# Autodesk Inventor assembly: Piston
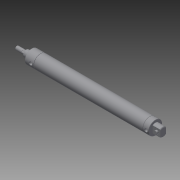
[picture p0: Inventor's stored thumbnail of the model, 180x180]
Saved by Autodesk Inventor 2014 (Build 180170000, 170)
## iProperties
Created: 2014-01-08
Part Number: Piston
Document SubType Name: Assembly
Designer: Tristan Debrunner
Author: Tristan Debrunner
## Documents named in this file (6)
- C:\Users\Tristan Debrunner\Documents\FRC 2014\Chassis\Piston.iam
- C:\Users\Tristan Debrunner\Documents\Inventor\Part2.ipt
- C:\Users\Tristan Debrunner\Documents\Inventor\Part4.ipt
- C:\Users\Tristan Debrunner\Documents\Inventor\Part6.ipt
- C:\Users\Tristan Debrunner\Documents\Inventor\Part8.ipt
- C:\Users\Tristan Debrunner\Documents\Inventor\Part10.ipt
## Components (5 placed, 5 different names)
1. Part2:1 — Mate:1
2. Part4:1
3. Part6:1
4. Part8:1
5. Part10:1 — Mate:1
## Relationships (1: Mate 1)
- Mate:1: Part2:1 ↔ Part10:1
